# Autodesk Inventor assembly: Cloud Chamber - Full Assembly
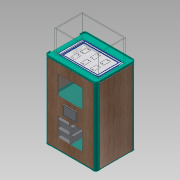
[picture p0: Inventor's stored thumbnail of the model, 180x180]
Saved by Autodesk Inventor 2015 (Build 190159000, 159)
## iProperties
Created: 2015-05-21
Part Number: Cloud Chamber - Full Assembly
Document SubType Name: Assembly
Designer: Joe Sheldon
Author: Joe Sheldon
## Documents named in this file (11)
- C:\Users\Joe Sheldon\Documents\PSU Stuff\PSU Clubs\Society of Physics Students\Cloud Chamber\Cloud Chamber CAD\Cloud Chamber - Full Assembly.iam
- C:\Users\Joe Sheldon\Documents\PSU Stuff\PSU Clubs\Society of Physics Students\Cloud Chamber\Cloud Chamber CAD\Cart\Cart_Chassis.iam
- C:\Users\Joe Sheldon\Documents\PSU Stuff\PSU Clubs\Society of Physics Students\Cloud Chamber\Cloud Chamber CAD\Cart\Panelling\cart_woodpanel-back.ipt
- C:\Users\Joe Sheldon\Documents\PSU Stuff\PSU Clubs\Society of Physics Students\Cloud Chamber\Cloud Chamber CAD\Cart\Panelling\cart_woodpanel-tall.ipt
- C:\Users\Joe Sheldon\Documents\PSU Stuff\PSU Clubs\Society of Physics Students\Cloud Chamber\Cloud Chamber CAD\Cart\Panelling\Front - Access\Front Panel.iam
- C:\Users\Joe Sheldon\Documents\PSU Stuff\PSU Clubs\Society of Physics Students\Cloud Chamber\Cloud Chamber CAD\Control System\User Control Panel - Rough.ipt
- C:\Users\Joe Sheldon\Documents\PSU Stuff\PSU Clubs\Society of Physics Students\Cloud Chamber\Cloud Chamber CAD\Power System\powersupply.ipt
- C:\Users\Joe Sheldon\Documents\PSU Stuff\PSU Clubs\Society of Physics Students\Cloud Chamber\Cloud Chamber CAD\Power System\power strip.ipt
- C:\Users\Joe Sheldon\Documents\PSU Stuff\PSU Clubs\Society of Physics Students\Cloud Chamber\Cloud Chamber CAD\Glass Tank\glass tank.ipt
- C:\Users\Joe Sheldon\Documents\PSU Stuff\PSU Clubs\Society of Physics Students\Cloud Chamber\Cloud Chamber CAD\Alcohol Flow System\Reservour - placeholder.ipt
- C:\Users\Joe Sheldon\Documents\PSU Stuff\PSU Clubs\Society of Physics Students\Cloud Chamber\Cloud Chamber CAD\MULTI-SYSTEM Assemblies\Cooling Plate and Catch Plate.iam
## Components (13 placed, 10 different names)
1. Cart_Chassis:1 [sub-assembly] — Rigid:1, Rigid:2, Rigid:3, Rigid:5, Rigid:6
2. cart_woodpanel-back:1 — Rigid:3
3. cart_woodpanel-tall:1 — Rigid:2
4. cart_woodpanel-tall:2 — Rigid:1
5. Front Panel:1 [sub-assembly] — Rigid:4, Rigid:5
6. User Control Panel - Rough:1 — Rigid:4
7. powersupply:1
8. powersupply:2
9. powersupply:3
10. power strip:1
11. glass tank:1 — Rigid:6
12. Reservour - placeholder:1
13. Cooling Plate and Catch Plate:1 [sub-assembly]
## Relationships (6: WeldJoint 6)
- Rigid:1 [WeldJoint]: Cart_Chassis:1 ↔ cart_woodpanel-tall:2
- Rigid:2 [WeldJoint]: Cart_Chassis:1 ↔ cart_woodpanel-tall:1
- Rigid:3 [WeldJoint]: Cart_Chassis:1 ↔ cart_woodpanel-back:1
- Rigid:4 [WeldJoint]: Front Panel:1 ↔ User Control Panel - Rough:1
- Rigid:5 [WeldJoint]: Cart_Chassis:1 ↔ Front Panel:1
- Rigid:6 [WeldJoint]: Cart_Chassis:1 ↔ glass tank:1
